# Autodesk Inventor assembly: Sestava1
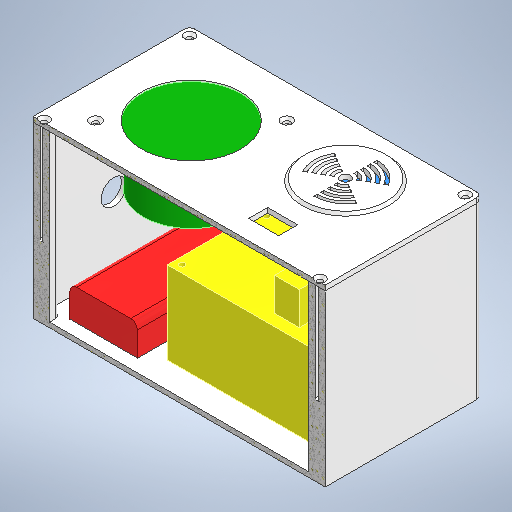
[picture p0: Inventor's stored thumbnail of the model, 512x512]
Saved by Autodesk Inventor 2025.2 (Build 292293000, 293)
## iProperties
Created: 2025-03-01
Part Number: Sestava1
Document SubType Name: Assembly
Designer: hepma_axt67em
Author: hepma_axt67em
## Documents named in this file (9)
- C:\Users\hepma_axt67em\Documents\Inventor\GeigerCounter\Sestava1.iam
- C:\Users\hepma_axt67em\Documents\Inventor\GeigerCounter\box_bottom.ipt
- C:\Users\hepma_axt67em\Documents\Inventor\GeigerCounter\prop_battery.ipt
- C:\Users\hepma_axt67em\Documents\Inventor\GeigerCounter\prop_meter.ipt
- C:\Users\hepma_axt67em\Documents\Inventor\GeigerCounter\prop_speaker.ipt
- C:\Users\hepma_axt67em\Documents\Inventor\GeigerCounter\prop_PCB.ipt
- C:\Users\hepma_axt67em\Documents\Inventor\GeigerCounter\box_top.ipt
- C:\Users\hepma_axt67em\Documents\Inventor\GeigerCounter\holder.ipt
- C:\Users\hepma_axt67em\Documents\Inventor\GeigerCounter\cover.ipt
## Components (8 placed, 8 different names)
1. box_bottom:1 — Proti sobě:1, Proti sobě:2, Proti sobě:3, Proti sobě:4, Proti sobě:5, Proti sobě:6, Proti sobě:7, Proti sobě:8, Proti sobě:11
2. prop_battery:1 — Proti sobě:1, Proti sobě:2, Proti sobě:3
3. prop_meter:1 — Proti sobě:9, Proti sobě:10, Proti sobě:15
4. prop_speaker:1 — Proti sobě:12, Proti sobě:13
5. prop_PCB:1 — Proti sobě:4, Proti sobě:5, Proti sobě:8
6. box_top:1 — Proti sobě:6, Proti sobě:7, Proti sobě:9, Proti sobě:10, Proti sobě:11, Proti sobě:12, Proti sobě:13, Proti sobě:16, Proti sobě:17, Proti sobě:18, Proti sobě:19
7. holder:1 — Proti sobě:15, Proti sobě:16, Proti sobě:17
8. cover:1 — Proti sobě:18, Proti sobě:19
## Relationships (18: Mate 18)
- Proti sobě:1 [Mate]: box_bottom:1 ↔ prop_battery:1
- Proti sobě:2 [Mate]: box_bottom:1 ↔ prop_battery:1
- Proti sobě:3 [Mate]: box_bottom:1 ↔ prop_battery:1
- Proti sobě:4 [Mate]: box_bottom:1 ↔ prop_PCB:1
- Proti sobě:5 [Mate]: box_bottom:1 ↔ prop_PCB:1
- Proti sobě:6 [Mate]: box_bottom:1 ↔ box_top:1
- Proti sobě:7 [Mate]: box_bottom:1 ↔ box_top:1
- Proti sobě:8 [Mate]: box_bottom:1 ↔ prop_PCB:1
- Proti sobě:9 [Mate]: prop_meter:1 ↔ box_top:1
- Proti sobě:10 [Mate]: prop_meter:1 ↔ box_top:1
- Proti sobě:11 [Mate]: box_bottom:1 ↔ box_top:1
- Proti sobě:12 [Mate]: prop_speaker:1 ↔ box_top:1
- Proti sobě:13 [Mate]: prop_speaker:1 ↔ box_top:1
- Proti sobě:15 [Mate]: prop_meter:1 ↔ holder:1
- Proti sobě:16 [Mate]: box_top:1 ↔ holder:1
- Proti sobě:17 [Mate]: box_top:1 ↔ holder:1
- Proti sobě:18 [Mate]: box_top:1 ↔ cover:1
- Proti sobě:19 [Mate]: box_top:1 ↔ cover:1
